# Autodesk Inventor assembly: WAGO Terminal Block
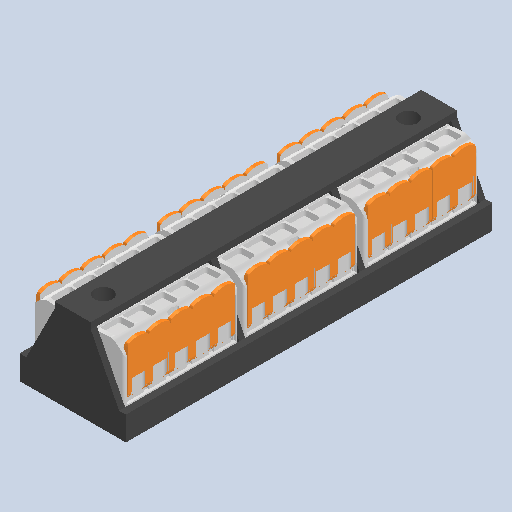
[picture p0: Inventor's stored thumbnail of the model, 512x512]
Saved by Autodesk Inventor 2024 (Build 280153000, 153)
## iProperties
Created: 2023-08-27
Part Number: WAGO Terminal Block
Document SubType Name: Assembly
Designer: 18179
Author: 18179
## Documents named in this file (3)
- C:\Users\18179\Desktop\TuppyMkIV_GitHub\TuppyMkIV\CAD\WAGO Terminal Block.iam
- C:\Users\18179\Desktop\TuppyMkIV_GitHub\TuppyMkIV\CAD\Wago mount.ipt
- C:\Users\18179\Desktop\TuppyMkIV_GitHub\TuppyMkIV\CAD\WAGO_5.ipt
## Components (7 placed, 2 different names)
1. Wago mount:1 — Mate:1, Mate:2, Mate:3, Mate:4, Mate:5, Mate:6, Mate:7, Mate:8, Mate:9, Mate:10, Mate:11, Mate:12, Mate:13, Mate:14, Mate:15, Mate:16, Mate:17, Mate:18
2. WAGO_5:1 — Mate:4, Mate:5, Mate:9
3. WAGO_5:2 — Mate:6, Mate:7, Mate:8
4. WAGO_5:3 — Mate:1, Mate:2, Mate:3
5. WAGO_5:4 — Mate:12, Mate:13, Mate:16
6. WAGO_5:5 — Mate:11, Mate:14, Mate:17
7. WAGO_5:6 — Mate:10, Mate:15, Mate:18
## Relationships (18: Mate 18)
- Mate:1: Wago mount:1 ↔ WAGO_5:3
- Mate:2: Wago mount:1 ↔ WAGO_5:3
- Mate:3: Wago mount:1 ↔ WAGO_5:3
- Mate:4: Wago mount:1 ↔ WAGO_5:1
- Mate:5: Wago mount:1 ↔ WAGO_5:1
- Mate:6: Wago mount:1 ↔ WAGO_5:2
- Mate:7: Wago mount:1 ↔ WAGO_5:2
- Mate:8: Wago mount:1 ↔ WAGO_5:2
- Mate:9: Wago mount:1 ↔ WAGO_5:1
- Mate:10: Wago mount:1 ↔ WAGO_5:6
- Mate:11: Wago mount:1 ↔ WAGO_5:5
- Mate:12: Wago mount:1 ↔ WAGO_5:4
- Mate:13: Wago mount:1 ↔ WAGO_5:4
- Mate:14: Wago mount:1 ↔ WAGO_5:5
- Mate:15: Wago mount:1 ↔ WAGO_5:6
- Mate:16: Wago mount:1 ↔ WAGO_5:4
- Mate:17: Wago mount:1 ↔ WAGO_5:5
- Mate:18: Wago mount:1 ↔ WAGO_5:6
